# Autodesk Inventor assembly: Сборка1
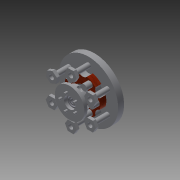
[picture p0: Inventor's stored thumbnail of the model, 180x180]
Saved by Autodesk Inventor 2013 (Build 170138000, 138)
## iProperties
Created: 2014-04-30
Part Number: Сборка1
Document SubType Name: Assembly
Designer: HP1
Author: HP1
## Documents named in this file (11)
- D:\##Цевочный редуктор\Сборка1.iam
- D:\##Цевочный редуктор\Статор цевков.ipt
- D:\##Цевочный редуктор\Сборка1\Мастер проектирования\Подшипник1.iam
- D:\##Цевочный редуктор\цевок10.ipt
- D:\##Цевочный редуктор\Ротор цевков.ipt
- D:\##Цевочный редуктор\ось.ipt
- D:\##Цевочный редуктор\ротор мотора.ipt
- D:\##Цевочный редуктор\статор мотора.ipt
- D:\##Цевочный редуктор\катушка.ipt
- D:\##Цевочный редуктор\ротор редуктора.ipt
- D:\##Цевочный редуктор\Сборка1\Мастер проектирования\Подшипник2.iam
## Components (20 placed, 9 different names)
1. Статор цевков:1 — Совмещение:1, Совмещение:2, Совмещение:3, Совмещение:4, Совмещение:5, Совмещение:6, Совмещение:7, Совмещение:8, Заподлицо:1, Заподлицо:2, Заподлицо:3, Заподлицо:4, Заподлицо:5, Заподлицо:6, Совмещение:17
2. Подшипник:1 [sub-assembly] — Совмещение:1, Совмещение:2, Совмещение:9, Совмещение:10
3. цевок10:1 — Совмещение:3, Заподлицо:4
4. цевок10:2 — Совмещение:4, Заподлицо:3
5. цевок10:3 — Совмещение:5, Заподлицо:2
6. цевок10:4 — Совмещение:6, Заподлицо:1
7. цевок10:5 — Совмещение:7, Заподлицо:6
8. цевок10:6 — Совмещение:8, Заподлицо:5, Совмещение:18
9. Ротор цевков:1 — Совмещение:11, Совмещение:12, Совмещение:13, Совмещение:14, Совмещение:15, Совмещение:27, Совмещение:28
10. ось:1 — Совмещение:9, Совмещение:10, Совмещение:11, Совмещение:12, Совмещение:16, Совмещение:25
11. ротор мотора:1 — Совмещение:13, Совмещение:14, Совмещение:15, Совмещение:26
12. статор мотора:1 — Совмещение:16, Совмещение:17, Совмещение:18, Совмещение:19, Заподлицо:7, Совмещение:20, Совмещение:21, Совмещение:22, Совмещение:23, Совмещение:24, Заподлицо:8, Заподлицо:9, Заподлицо:10, Заподлицо:11, Заподлицо:12
13. катушка:1 — Совмещение:19, Заподлицо:7
14. катушка:2 — Совмещение:20, Заподлицо:8
15. катушка:3 — Совмещение:21, Заподлицо:9
16. катушка:4 — Совмещение:22, Заподлицо:10
17. катушка:5 — Совмещение:23, Заподлицо:11
18. катушка:6 — Совмещение:24, Заподлицо:12
19. ротор редуктора:1 — Совмещение:25, Совмещение:26
20. Подшипник:2 [sub-assembly] — Совмещение:27, Совмещение:28
## Relationships (40: Mate 28, Flush 12)
- Совмещение:1 [Mate]: Статор цевков:1 ↔ Подшипник:1
- Совмещение:2 [Mate]: Статор цевков:1 ↔ Подшипник:1
- Совмещение:3 [Mate]: Статор цевков:1 ↔ цевок10:1
- Совмещение:4 [Mate]: Статор цевков:1 ↔ цевок10:2
- Совмещение:5 [Mate]: Статор цевков:1 ↔ цевок10:3
- Совмещение:6 [Mate]: Статор цевков:1 ↔ цевок10:4
- Совмещение:7 [Mate]: Статор цевков:1 ↔ цевок10:5
- Совмещение:8 [Mate]: Статор цевков:1 ↔ цевок10:6
- Заподлицо:1 [Flush]: Статор цевков:1 ↔ цевок10:4
- Заподлицо:2 [Flush]: Статор цевков:1 ↔ цевок10:3
- Заподлицо:3 [Flush]: Статор цевков:1 ↔ цевок10:2
- Заподлицо:4 [Flush]: Статор цевков:1 ↔ цевок10:1
- Заподлицо:5 [Flush]: Статор цевков:1 ↔ цевок10:6
- Заподлицо:6 [Flush]: Статор цевков:1 ↔ цевок10:5
- Совмещение:9 [Mate]: Подшипник:1 ↔ ось:1
- Совмещение:10 [Mate]: Подшипник:1 ↔ ось:1
- Совмещение:11 [Mate]: Ротор цевков:1 ↔ ось:1
- Совмещение:12 [Mate]: Ротор цевков:1 ↔ ось:1
- Совмещение:13 [Mate]: Ротор цевков:1 ↔ ротор мотора:1
- Совмещение:14 [Mate]: Ротор цевков:1 ↔ ротор мотора:1
- Совмещение:15 [Mate]: Ротор цевков:1 ↔ ротор мотора:1
- Совмещение:16 [Mate]: ось:1 ↔ статор мотора:1
- Совмещение:17 [Mate]: Статор цевков:1 ↔ статор мотора:1
- Совмещение:18 [Mate]: цевок10:6 ↔ статор мотора:1
- Совмещение:19 [Mate]: статор мотора:1 ↔ катушка:1
- Заподлицо:7 [Flush]: статор мотора:1 ↔ катушка:1
- Совмещение:20 [Mate]: статор мотора:1 ↔ катушка:2
- Совмещение:21 [Mate]: статор мотора:1 ↔ катушка:3
- Совмещение:22 [Mate]: статор мотора:1 ↔ катушка:4
- Совмещение:23 [Mate]: статор мотора:1 ↔ катушка:5
- Совмещение:24 [Mate]: статор мотора:1 ↔ катушка:6
- Заподлицо:8 [Flush]: статор мотора:1 ↔ катушка:2
- Заподлицо:9 [Flush]: статор мотора:1 ↔ катушка:3
- Заподлицо:10 [Flush]: статор мотора:1 ↔ катушка:4
- Заподлицо:11 [Flush]: статор мотора:1 ↔ катушка:5
- Совмещение:25 [Mate]: ось:1 ↔ ротор редуктора:1
- Совмещение:26 [Mate] (1 mm): ротор мотора:1 ↔ ротор редуктора:1
- Заподлицо:12 [Flush]: статор мотора:1 ↔ катушка:6
- Совмещение:27 [Mate]: Ротор цевков:1 ↔ Подшипник:2
- Совмещение:28 [Mate]: Ротор цевков:1 ↔ Подшипник:2
